# Autodesk Inventor assembly: Frame 1647030135921
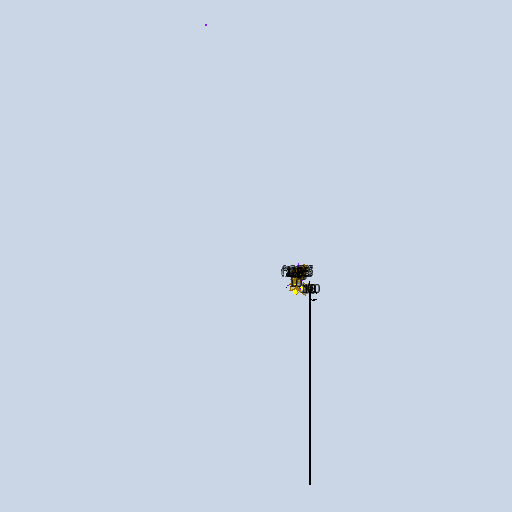
[picture p0: Inventor's stored thumbnail of the model, 512x512]
Saved by Autodesk Inventor 2022.2 (Build 262287000, 287)
## iProperties
_FrameDoc: Frame Assembly
_Version: 25.0.0
Created: 2022-03-11
Part Number: Frame 1647030135921
Document SubType Name: Assembly
Designer: foriw
Mass: 6891.58 g
Surface Area: 9076.06 cm^2
Volume: 2305.1 cm^3
Density: 2.98971 g/cm^3
Author: foriw
## Documents named in this file (28)
- H:\inventor ting\Mekatronik beercart git\Beercart CAD\Workspaces\Workspace\beercart assembly - mekatronik\Frame\Frame 1647030135921.iam
- H:\inventor ting\Mekatronik beercart git\Beercart CAD\Workspaces\Workspace\beercart assembly - mekatronik\Frame\Skeleton 1647030135922.ipt
- H:\inventor ting\Mekatronik beercart git\Beercart CAD\Workspaces\Workspace\beercart assembly - mekatronik\Frame\ISO 12633-2 20x20x2 1647030639616.ipt
- H:\inventor ting\Mekatronik beercart git\Beercart CAD\Workspaces\Workspace\beercart assembly - mekatronik\Frame\ISO 12633-2 20x20x2 1647030639707.ipt
- H:\inventor ting\Mekatronik beercart git\Beercart CAD\Workspaces\Workspace\beercart assembly - mekatronik\Frame\ISO 12633-2 20x20x2 1647606177438.ipt
- H:\inventor ting\Mekatronik beercart git\Beercart CAD\Workspaces\Workspace\BackWheelMountingPlate.ipt
- H:\inventor ting\Mekatronik beercart git\Beercart CAD\Workspaces\Workspace\beercart assembly - mekatronik\Frame\ISO 12633-2 20x20x2 1648573909221.ipt
- H:\inventor ting\Mekatronik beercart git\Beercart CAD\Workspaces\Workspace\beercart assembly - mekatronik\Frame\ISO 12633-2 20x20x2 1648573975084.ipt
- H:\inventor ting\Mekatronik beercart git\Beercart CAD\Workspaces\Workspace\beercart assembly - mekatronik\Frame\ISO 12633-2 20x20x2 1648627088055.ipt
- H:\inventor ting\Mekatronik beercart git\Beercart CAD\Workspaces\Workspace\beercart assembly - mekatronik\Frame\ISO 12633-2 20x20x2 1648627088175.ipt
- H:\inventor ting\Mekatronik beercart git\Beercart CAD\Workspaces\Workspace\BackWheelMountingPlate_MIR4.ipt
- H:\inventor ting\Mekatronik beercart git\Beercart CAD\Workspaces\Workspace\beercart assembly - mekatronik\Frame\ISO 12633-2 20x20x2 1649085652950.ipt
- H:\inventor ting\Mekatronik beercart git\Beercart CAD\Workspaces\Workspace\beercart assembly - mekatronik\Frame\ISO 12633-2 20x20x2 1649085653040.ipt
- H:\inventor ting\Mekatronik beercart git\Beercart CAD\Workspaces\Workspace\backWheelNoMotor brake mount.ipt
- H:\inventor ting\Mekatronik beercart git\Beercart CAD\Workspaces\Workspace\beercart assembly - mekatronik\Frame\ISO 12633-2 20x20x2 1649154464355.ipt
- H:\inventor ting\Mekatronik beercart git\Beercart CAD\Workspaces\Workspace\BackWheelMotorMountSpacer.ipt
- H:\inventor ting\Mekatronik beercart git\Beercart CAD\Workspaces\Workspace\beercart assembly - mekatronik\Frame\FrontWheelFrameNew.iam
- H:\inventor ting\Mekatronik beercart git\Beercart CAD\Workspaces\Workspace\headset bearing.ipt
- H:\inventor ting\Mekatronik beercart git\Beercart CAD\Workspaces\Workspace\beercart assembly - mekatronik\Frame\ISO 12633-2 20x20x2 1650129877673.ipt
- H:\inventor ting\Mekatronik beercart git\Beercart CAD\Workspaces\Workspace\beercart assembly - mekatronik\Frame\ISO 12633-2 20x20x2 1650129879551.ipt
- H:\inventor ting\Mekatronik beercart git\Beercart CAD\Workspaces\Workspace\beercart assembly - mekatronik\Frame\ISO 12633-2 20x20x2 1650129879650.ipt
- H:\inventor ting\Mekatronik beercart git\Beercart CAD\Workspaces\Workspace\beercart assembly - mekatronik\Frame\ISO 12633-2 20x20x2 1650129879749.ipt
- H:\inventor ting\Mekatronik beercart git\Beercart CAD\Workspaces\Workspace\beercart assembly - mekatronik\Frame\ISO 12633-2 20x20x2 1650134807858.ipt
- H:\inventor ting\Mekatronik beercart git\Beercart CAD\Workspaces\Workspace\beercart assembly - mekatronik\Frame\plan1 .iam
- H:\inventor ting\Mekatronik beercart git\Beercart CAD\Workspaces\Workspace\beercart assembly - mekatronik\Frame\Plan 2 øverste.iam
- H:\inventor ting\Mekatronik beercart git\Beercart CAD\Workspaces\Workspace\beercart assembly - mekatronik\Frame\GlidelejrehusAssembly.iam
- H:\inventor ting\Mekatronik beercart git\Beercart CAD\Libraries\Content Center Files\en-US\ISO 4762(2)\ISO 4762 - M6 x 50ISO.ipt
- H:\inventor ting\Mekatronik beercart git\Beercart CAD\Libraries\Content Center Files\en-US\ISO 7041\ISO 7041 - M6 - ISO.ipt
## Components (34 placed, 24 different names)
1. Reference Skeleton
2. ISO 12633-2 20x20x2 - 250,13:1
3. ISO 12633-2 20x20x2 - 250,13:2
4. ISO 12633-2 20x20x2 - 123,73:2 — Mate:2, Mate:4, Mate:5
5. BackWheelMountingPlate:1 — Flush:6, Rotational:2, Rigid:1
6. ISO 12633-2 20x20x2 - 360,44:1
7. ISO 12633-2 20x20x2 - plan1 left wheel mount — Flush:6, Rotational:2, Rigid:1
8. ISO 12633-2 20x20x2 - 107,97:1 — Flush:9, Flush:11, Flush:12, Flush:13, Rigid:2
9. ISO 12633-2 20x20x2 - 115.41:1
10. BackWheelMountingPlate_MIR4:1 — Flush:9, Rigid:2
11. ISO 12633-2 20x20x2 - 120.65:1 — Flush:14
12. ISO 12633-2 20x20x2 - 113,38:1 — Flush:10
13. backWheelNoMotor brake mount:1 — Flush:10, Flush:14
14. ISO 12633-2 20x20x2 - plan1 right wheel mount
15. BackWheelMotorMountSpacer:1 — Flush:11, Flush:12, Flush:13
16. FrontWheelFrameNew:1 [sub-assembly] — Insert:3, Insert:4
17. headset bearing:1 — Insert:3
18. ISO 12633-2 20x20x2 - 76,3:1
19. ISO 12633-2 20x20x2 - 85,41:1 — Mate:28, Mate:30, Mate:31, Mate:32, Mate:34, Mate:35
20. ISO 12633-2 20x20x2 - 85,41:2 — Rigid:3, Mate:39, Mate:40, Mate:42, Mate:43
21. ISO 12633-2 20x20x2 - 76,3:2 — Mate:36, Mate:38
22. ISO 12633-2 20x20x2 - 98,29:1
23. plan1 højre :1 [sub-assembly]
24. Plan 2 øverste:1 [sub-assembly]
25. GlidelejrehusAssembly:1 [sub-assembly] — Insert:4, Mate:29, Mate:33
26. GlidelejrehusAssembly:2 [sub-assembly] — Rigid:3, Mate:37, Mate:41
27. ISO 4762 M6 x 50:1 — Mate:28, Mate:29
28. ISO 7041 M6:1 — Mate:30, Mate:31
29. ISO 4762 M6 x 50:2 — Mate:32, Mate:33
30. ISO 7041 M6:2 — Mate:34, Mate:35
31. ISO 4762 M6 x 50:3 — Mate:36, Mate:37
32. ISO 7041 M6:3 — Mate:38, Mate:39
33. ISO 4762 M6 x 50:4 — Mate:40, Mate:41
34. ISO 7041 M6:4 — Mate:42, Mate:43
## Relationships (35: Mate 21, Flush 8, WeldJoint 3, Insert 2, RevoluteJoint 1)
- Mate:2: ISO 12633-2 20x20x2 - 123,73:2
- Mate:4: ISO 12633-2 20x20x2 - 123,73:2
- Mate:5: ISO 12633-2 20x20x2 - 123,73:2
- Flush:6: BackWheelMountingPlate:1 ↔ ISO 12633-2 20x20x2 - plan1 left wheel mount
- Rotational:2 [RevoluteJoint]: BackWheelMountingPlate:1 ↔ ISO 12633-2 20x20x2 - plan1 left wheel mount
- Flush:9: ISO 12633-2 20x20x2 - 107,97:1 ↔ BackWheelMountingPlate_MIR4:1
- Flush:10: ISO 12633-2 20x20x2 - 113,38:1 ↔ backWheelNoMotor brake mount:1
- Rigid:1 [WeldJoint]: BackWheelMountingPlate:1 ↔ ISO 12633-2 20x20x2 - plan1 left wheel mount
- Flush:11: ISO 12633-2 20x20x2 - 107,97:1 ↔ BackWheelMotorMountSpacer:1
- Flush:12: ISO 12633-2 20x20x2 - 107,97:1 ↔ BackWheelMotorMountSpacer:1
- Flush:13: ISO 12633-2 20x20x2 - 107,97:1 ↔ BackWheelMotorMountSpacer:1
- Flush:14: ISO 12633-2 20x20x2 - 120.65:1 ↔ backWheelNoMotor brake mount:1
- Insert:3: FrontWheelFrameNew:1 ↔ headset bearing:1
- Rigid:2 [WeldJoint]: ISO 12633-2 20x20x2 - 107,97:1 ↔ BackWheelMountingPlate_MIR4:1
- [Flush]: ISO 12633-2 20x20x2 - 85,41:1 ↔ GlidelejrehusAssembly:1
- [Mate]: FrontWheelFrameNew:1 ↔ GlidelejrehusAssembly:1
- [Mate]: ISO 12633-2 20x20x2 - 85,41:1 ↔ GlidelejrehusAssembly:1
- Rigid:3 [WeldJoint]: ISO 12633-2 20x20x2 - 85,41:2 ↔ GlidelejrehusAssembly:2
- Insert:4: FrontWheelFrameNew:1 ↔ GlidelejrehusAssembly:1
- Mate:28: ISO 12633-2 20x20x2 - 85,41:1 ↔ ISO 4762 M6 x 50:1
- Mate:29: GlidelejrehusAssembly:1 ↔ ISO 4762 M6 x 50:1
- Mate:30: ISO 12633-2 20x20x2 - 85,41:1 ↔ ISO 7041 M6:1
- Mate:31: ISO 12633-2 20x20x2 - 85,41:1 ↔ ISO 7041 M6:1
- Mate:32: ISO 12633-2 20x20x2 - 85,41:1 ↔ ISO 4762 M6 x 50:2
- Mate:33: GlidelejrehusAssembly:1 ↔ ISO 4762 M6 x 50:2
- Mate:34: ISO 12633-2 20x20x2 - 85,41:1 ↔ ISO 7041 M6:2
- Mate:35: ISO 12633-2 20x20x2 - 85,41:1 ↔ ISO 7041 M6:2
- Mate:36: ISO 12633-2 20x20x2 - 76,3:2 ↔ ISO 4762 M6 x 50:3
- Mate:37: GlidelejrehusAssembly:2 ↔ ISO 4762 M6 x 50:3
- Mate:38: ISO 12633-2 20x20x2 - 76,3:2 ↔ ISO 7041 M6:3
- Mate:39: ISO 12633-2 20x20x2 - 85,41:2 ↔ ISO 7041 M6:3
- Mate:40: ISO 12633-2 20x20x2 - 85,41:2 ↔ ISO 4762 M6 x 50:4
- Mate:41: GlidelejrehusAssembly:2 ↔ ISO 4762 M6 x 50:4
- Mate:42: ISO 12633-2 20x20x2 - 85,41:2 ↔ ISO 7041 M6:4
- Mate:43: ISO 12633-2 20x20x2 - 85,41:2 ↔ ISO 7041 M6:4
